# Autodesk Inventor assembly: Assembly
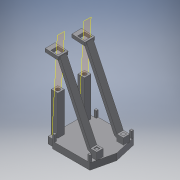
[picture p0: Inventor's stored thumbnail of the model, 180x180]
Saved by Autodesk Inventor 2016 (Build 200138000, 138)
## iProperties
Created: 2018-01-06
Part Number: Assembly
Document SubType Name: Assembly
Designer: Jorian Bruslind
Author: Jorian Bruslind
## Documents named in this file (3)
- C:\Users\Jorian Bruslind\Documents\GitHub\PersonalProjects\Inventor Projects\Maglev\Assembly.iam
- C:\Users\Jorian Bruslind\Documents\GitHub\PersonalProjects\Inventor Projects\Maglev\Maglev_Stand.ipt
- C:\Users\Jorian Bruslind\Documents\GitHub\PersonalProjects\Inventor Projects\Maglev\Maglev_supports.ipt
## Components (3 placed, 2 different names)
1. Maglev_Stand:1 — Mate:1, Mate:2, Mate:3, Flush:1, Mate:4
2. Maglev_supports:1 — Mate:1, Mate:2
3. Maglev_supports:2 — Mate:3, Flush:1, Mate:4
## Relationships (5: Mate 4, Flush 1)
- Mate:1: Maglev_Stand:1 ↔ Maglev_supports:1
- Mate:2: Maglev_Stand:1 ↔ Maglev_supports:1
- Mate:3: Maglev_Stand:1 ↔ Maglev_supports:2
- Flush:1: Maglev_Stand:1 ↔ Maglev_supports:2
- Mate:4: Maglev_Stand:1 ↔ Maglev_supports:2
